# Autodesk Inventor assembly: Cabinet-LogicCircuit
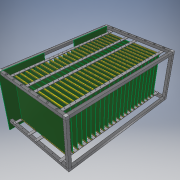
[picture p0: Inventor's stored thumbnail of the model, 180x180]
Saved by Autodesk Inventor 2018 (Build 220112000, 112)
## iProperties
Created: 2025-02-17
Part Number: Cabinet-LogicCircuit
Material: Všeobecné
Document SubType Name: Assembly
Designer: Jozko Mrkvicka
Author: Jozko Mrkvicka
## Documents named in this file (11)
- D:\05_Projekty\Projects_Inventor\Haluska9000\Cabinet-LogicCircuit.iam
- D:\05_Projekty\Projects_Inventor\Haluska9000\Profile-Connector.ipt
- D:\05_Projekty\Projects_Inventor\Haluska9000\Profile-Connector\Profile-Connector#15x15xCorner.ipt
- D:\05_Projekty\Projects_Inventor\Haluska9000\PCB.ipt
- D:\05_Projekty\Projects_Inventor\Haluska9000\CardGuideArray-4-Inch.iam
- D:\05_Projekty\Projects_Inventor\Haluska9000\CardGuideArray-6-Inch.iam
- D:\05_Projekty\Projects_Inventor\Haluska9000\Profile-Square-Gray\Profile-Square#Cabinet-LogicCircuit-Width.ipt
- D:\05_Projekty\Projects_Inventor\Haluska9000\Profile-Square-Gray\Profile-Square#Cabinet-LogicCircuit-Height.ipt
- D:\05_Projekty\Projects_Inventor\Haluska9000\Profile-Square-Gray\Profile-Square#Cabinet-LogicCircuit-Length.ipt
- D:\05_Projekty\Projects_Inventor\Haluska9000\Profile-Square-Gray.ipt
- D:\05_Projekty\Projects_Inventor\Haluska9000\PCB\PCB#LogicCircuit.ipt
## Components (49 placed, 8 different names)
1. Profile-Square#Cabinet-LogicCircuit-Width:15
2. Profile-Square#Cabinet-LogicCircuit-Width:18
3. Profile-Square#Cabinet-LogicCircuit-Width:21
4. Profile-Square#Cabinet-LogicCircuit-Width:24
5. Profile-Square#Cabinet-LogicCircuit-Height:14
6. Profile-Square#Cabinet-LogicCircuit-Height:17
7. Profile-Square#Cabinet-LogicCircuit-Height:20
8. Profile-Square#Cabinet-LogicCircuit-Height:23
9. Profile-Square#Cabinet-LogicCircuit-Length:13 — Stejný směr:152, Stejný směr:153, Proti sobě:353, Proti sobě:354, Proti sobě:356, Proti sobě:357
10. Profile-Square#Cabinet-LogicCircuit-Length:16 — Proti sobě:360, Proti sobě:361, Stejný směr:399, Stejný směr:400, Proti sobě:362, Proti sobě:363
11. Profile-Square#Cabinet-LogicCircuit-Length:19
12. Profile-Square#Cabinet-LogicCircuit-Length:22
13. Profile-Connector#15x15xCorner:17
14. Profile-Connector#15x15xCorner:18
15. Profile-Connector#15x15xCorner:19
16. Profile-Connector#15x15xCorner:20
17. Profile-Connector#15x15xCorner:21
18. Profile-Connector#15x15xCorner:22
19. Profile-Connector#15x15xCorner:23
20. Profile-Connector#15x15xCorner:24
21. PCB:19
22. PCB:20
23. CardGuideArray-4-Inch:1 [sub-assembly] — Stejný směr:152, Proti sobě:354, Proti sobě:357
24. CardGuideArray-6-Inch:1 [sub-assembly] — Stejný směr:153, Proti sobě:353, Proti sobě:356, Proti sobě:358, Proti sobě:359
25. PCB#LogicCircuit:1 — Stejný směr:154, Stejný směr:176, Stejný směr:360, Proti sobě:358, Proti sobě:359
26. PCB#LogicCircuit:2 — Stejný směr:154, Stejný směr:155, Stejný směr:176, Stejný směr:177, Stejný směr:360, Stejný směr:361
27. PCB#LogicCircuit:3 — Stejný směr:155, Stejný směr:156, Stejný směr:177, Stejný směr:178, Stejný směr:361, Stejný směr:362
28. PCB#LogicCircuit:4 — Stejný směr:156, Stejný směr:157, Stejný směr:178, Stejný směr:179, Stejný směr:362, Stejný směr:363
29. PCB#LogicCircuit:5 — Stejný směr:157, Stejný směr:158, Stejný směr:179, Stejný směr:359, Stejný směr:363, Stejný směr:364
30. PCB#LogicCircuit:6 — Stejný směr:158, Stejný směr:159, Stejný směr:359, Stejný směr:381, Stejný směr:364, Stejný směr:397
31. PCB#LogicCircuit:7 — Stejný směr:159, Stejný směr:160, Stejný směr:381, Stejný směr:365, Stejný směr:382, Stejný směr:397
32. PCB#LogicCircuit:8 — Stejný směr:160, Stejný směr:161, Stejný směr:365, Stejný směr:366, Stejný směr:382, Stejný směr:383
33. PCB#LogicCircuit:9 — Stejný směr:161, Stejný směr:162, Stejný směr:366, Stejný směr:367, Stejný směr:383, Stejný směr:384
34. PCB#LogicCircuit:10 — Stejný směr:162, Stejný směr:163, Stejný směr:367, Stejný směr:368, Stejný směr:384, Stejný směr:385
35. PCB#LogicCircuit:11 — Stejný směr:163, Stejný směr:164, Stejný směr:368, Stejný směr:369, Stejný směr:385, Stejný směr:386
36. PCB#LogicCircuit:12 — Stejný směr:164, Stejný směr:165, Stejný směr:369, Stejný směr:370, Stejný směr:386, Stejný směr:387
37. PCB#LogicCircuit:13 — Stejný směr:165, Stejný směr:166, Stejný směr:370, Stejný směr:371, Stejný směr:387, Stejný směr:388
38. PCB#LogicCircuit:14 — Stejný směr:166, Stejný směr:167, Stejný směr:371, Stejný směr:372, Stejný směr:388, Stejný směr:389
39. PCB#LogicCircuit:15 — Stejný směr:167, Stejný směr:168, Stejný směr:372, Stejný směr:373, Stejný směr:389, Stejný směr:390
40. PCB#LogicCircuit:16 — Stejný směr:168, Stejný směr:169, Stejný směr:373, Stejný směr:374, Stejný směr:390, Stejný směr:391
41. PCB#LogicCircuit:17 — Stejný směr:169, Stejný směr:170, Stejný směr:374, Stejný směr:375, Stejný směr:391, Stejný směr:392
42. PCB#LogicCircuit:18 — Stejný směr:170, Stejný směr:171, Stejný směr:375, Stejný směr:376, Stejný směr:392, Stejný směr:398
43. PCB#LogicCircuit:19 — Stejný směr:171, Stejný směr:172, Stejný směr:376, Stejný směr:377, Stejný směr:393, Stejný směr:398
44. PCB#LogicCircuit:20 — Stejný směr:172, Stejný směr:173, Stejný směr:377, Stejný směr:378, Stejný směr:393, Stejný směr:394
45. PCB#LogicCircuit:21 — Stejný směr:173, Stejný směr:174, Stejný směr:378, Stejný směr:379, Stejný směr:394, Stejný směr:395
46. PCB#LogicCircuit:22 — Stejný směr:174, Stejný směr:175, Stejný směr:379, Stejný směr:380, Stejný směr:395, Stejný směr:396
47. PCB#LogicCircuit:23 — Stejný směr:175, Stejný směr:380, Stejný směr:396
48. CardGuideArray-4-Inch:2 [sub-assembly] — Proti sobě:360, Stejný směr:399, Proti sobě:362
49. CardGuideArray-6-Inch:2 [sub-assembly] — Proti sobě:361, Stejný směr:400, Proti sobě:363
## Relationships (143: Flush 72, Mate 71)
- [Mate]: Profile-Square#Cabinet-LogicCircuit-Length:13 ↔ Profile-Connector#15x15xCorner:17
- [Mate]: Profile-Square#Cabinet-LogicCircuit-Length:13 ↔ Profile-Connector#15x15xCorner:17
- [Mate]: Profile-Square#Cabinet-LogicCircuit-Length:13 ↔ Profile-Connector#15x15xCorner:17
- [Mate]: Profile-Square#Cabinet-LogicCircuit-Height:14 ↔ Profile-Connector#15x15xCorner:17
- [Mate]: Profile-Square#Cabinet-LogicCircuit-Height:14 ↔ Profile-Connector#15x15xCorner:17
- [Mate]: Profile-Square#Cabinet-LogicCircuit-Height:14 ↔ Profile-Connector#15x15xCorner:17
- [Mate]: Profile-Square#Cabinet-LogicCircuit-Width:15 ↔ Profile-Connector#15x15xCorner:17
- [Mate]: Profile-Square#Cabinet-LogicCircuit-Width:15 ↔ Profile-Connector#15x15xCorner:17
- [Mate]: Profile-Square#Cabinet-LogicCircuit-Width:15 ↔ Profile-Connector#15x15xCorner:17
- [Mate]: Profile-Square#Cabinet-LogicCircuit-Length:13 ↔ Profile-Connector#15x15xCorner:18
- [Mate]: Profile-Square#Cabinet-LogicCircuit-Length:13 ↔ Profile-Connector#15x15xCorner:18
- [Mate]: Profile-Square#Cabinet-LogicCircuit-Length:13 ↔ Profile-Connector#15x15xCorner:18
- [Mate]: Profile-Square#Cabinet-LogicCircuit-Length:16 ↔ Profile-Connector#15x15xCorner:19
- [Mate]: Profile-Square#Cabinet-LogicCircuit-Length:16 ↔ Profile-Connector#15x15xCorner:19
- [Mate]: Profile-Square#Cabinet-LogicCircuit-Length:16 ↔ Profile-Connector#15x15xCorner:19
- [Mate]: Profile-Square#Cabinet-LogicCircuit-Height:17 ↔ Profile-Connector#15x15xCorner:19
- [Mate]: Profile-Square#Cabinet-LogicCircuit-Height:17 ↔ Profile-Connector#15x15xCorner:19
- [Mate]: Profile-Square#Cabinet-LogicCircuit-Height:17 ↔ Profile-Connector#15x15xCorner:19
- [Mate]: Profile-Square#Cabinet-LogicCircuit-Width:18 ↔ Profile-Connector#15x15xCorner:19
- [Mate]: Profile-Square#Cabinet-LogicCircuit-Width:18 ↔ Profile-Connector#15x15xCorner:19
- [Mate]: Profile-Square#Cabinet-LogicCircuit-Width:18 ↔ Profile-Connector#15x15xCorner:19
- [Mate]: Profile-Square#Cabinet-LogicCircuit-Length:16 ↔ Profile-Connector#15x15xCorner:20
- [Mate]: Profile-Square#Cabinet-LogicCircuit-Length:16 ↔ Profile-Connector#15x15xCorner:20
- [Mate]: Profile-Square#Cabinet-LogicCircuit-Length:16 ↔ Profile-Connector#15x15xCorner:20
- [Mate]: Profile-Square#Cabinet-LogicCircuit-Height:17 ↔ Profile-Connector#15x15xCorner:18
- [Mate]: Profile-Square#Cabinet-LogicCircuit-Height:17 ↔ Profile-Connector#15x15xCorner:18
- [Mate]: Profile-Square#Cabinet-LogicCircuit-Height:17 ↔ Profile-Connector#15x15xCorner:18
- [Mate]: Profile-Square#Cabinet-LogicCircuit-Length:19 ↔ Profile-Connector#15x15xCorner:21
- [Mate]: Profile-Square#Cabinet-LogicCircuit-Length:19 ↔ Profile-Connector#15x15xCorner:21
- [Mate]: Profile-Square#Cabinet-LogicCircuit-Length:19 ↔ Profile-Connector#15x15xCorner:21
- [Mate]: Profile-Square#Cabinet-LogicCircuit-Height:20 ↔ Profile-Connector#15x15xCorner:21
- [Mate]: Profile-Square#Cabinet-LogicCircuit-Height:20 ↔ Profile-Connector#15x15xCorner:21
- [Mate]: Profile-Square#Cabinet-LogicCircuit-Height:20 ↔ Profile-Connector#15x15xCorner:21
- [Mate]: Profile-Square#Cabinet-LogicCircuit-Width:21 ↔ Profile-Connector#15x15xCorner:21
- [Mate]: Profile-Square#Cabinet-LogicCircuit-Width:21 ↔ Profile-Connector#15x15xCorner:21
- [Mate]: Profile-Square#Cabinet-LogicCircuit-Width:21 ↔ Profile-Connector#15x15xCorner:21
- [Mate]: Profile-Square#Cabinet-LogicCircuit-Length:19 ↔ Profile-Connector#15x15xCorner:22
- [Mate]: Profile-Square#Cabinet-LogicCircuit-Length:19 ↔ Profile-Connector#15x15xCorner:22
- [Mate]: Profile-Square#Cabinet-LogicCircuit-Length:19 ↔ Profile-Connector#15x15xCorner:22
- [Mate]: Profile-Square#Cabinet-LogicCircuit-Length:22 ↔ Profile-Connector#15x15xCorner:23
- [Mate]: Profile-Square#Cabinet-LogicCircuit-Length:22 ↔ Profile-Connector#15x15xCorner:23
- [Mate]: Profile-Square#Cabinet-LogicCircuit-Length:22 ↔ Profile-Connector#15x15xCorner:23
- [Mate]: Profile-Square#Cabinet-LogicCircuit-Height:23 ↔ Profile-Connector#15x15xCorner:23
- [Mate]: Profile-Square#Cabinet-LogicCircuit-Height:23 ↔ Profile-Connector#15x15xCorner:23
- [Mate]: Profile-Square#Cabinet-LogicCircuit-Height:23 ↔ Profile-Connector#15x15xCorner:23
- [Mate]: Profile-Square#Cabinet-LogicCircuit-Width:24 ↔ Profile-Connector#15x15xCorner:23
- [Mate]: Profile-Square#Cabinet-LogicCircuit-Width:24 ↔ Profile-Connector#15x15xCorner:23
- [Mate]: Profile-Square#Cabinet-LogicCircuit-Width:24 ↔ Profile-Connector#15x15xCorner:23
- [Mate]: Profile-Square#Cabinet-LogicCircuit-Length:22 ↔ Profile-Connector#15x15xCorner:24
- [Mate]: Profile-Square#Cabinet-LogicCircuit-Length:22 ↔ Profile-Connector#15x15xCorner:24
- [Mate]: Profile-Square#Cabinet-LogicCircuit-Length:22 ↔ Profile-Connector#15x15xCorner:24
- [Mate]: Profile-Square#Cabinet-LogicCircuit-Height:23 ↔ Profile-Connector#15x15xCorner:22
- [Mate]: Profile-Square#Cabinet-LogicCircuit-Height:23 ↔ Profile-Connector#15x15xCorner:22
- [Mate]: Profile-Square#Cabinet-LogicCircuit-Height:23 ↔ Profile-Connector#15x15xCorner:22
- [Mate]: Profile-Square#Cabinet-LogicCircuit-Width:21 ↔ Profile-Connector#15x15xCorner:18
- [Mate]: Profile-Square#Cabinet-LogicCircuit-Width:21 ↔ Profile-Connector#15x15xCorner:18
- [Mate]: Profile-Square#Cabinet-LogicCircuit-Width:21 ↔ Profile-Connector#15x15xCorner:18
- [Flush]: Profile-Square#Cabinet-LogicCircuit-Width:18 ↔ PCB:19
- [Mate]: Profile-Square#Cabinet-LogicCircuit-Width:18 ↔ PCB:19
- [Mate]: Profile-Square#Cabinet-LogicCircuit-Length:16 ↔ PCB:19
- [Mate]: Profile-Square#Cabinet-LogicCircuit-Width:18 ↔ PCB:20
- [Flush]: Profile-Square#Cabinet-LogicCircuit-Width:18 ↔ PCB:20
- [Mate]: Profile-Square#Cabinet-LogicCircuit-Length:22 ↔ PCB:20
- Stejný směr:152 [Flush]: Profile-Square#Cabinet-LogicCircuit-Length:13 ↔ CardGuideArray-4-Inch:1
- Stejný směr:153 [Flush]: Profile-Square#Cabinet-LogicCircuit-Length:13 ↔ CardGuideArray-6-Inch:1
- Proti sobě:353 [Mate]: Profile-Square#Cabinet-LogicCircuit-Length:13 ↔ CardGuideArray-6-Inch:1
- Proti sobě:354 [Mate]: Profile-Square#Cabinet-LogicCircuit-Length:13 ↔ CardGuideArray-4-Inch:1
- Proti sobě:356 [Mate]: Profile-Square#Cabinet-LogicCircuit-Length:13 ↔ CardGuideArray-6-Inch:1
- Proti sobě:357 [Mate]: Profile-Square#Cabinet-LogicCircuit-Length:13 ↔ CardGuideArray-4-Inch:1
- Stejný směr:154 [Flush] (25.4 mm): PCB#LogicCircuit:1 ↔ PCB#LogicCircuit:2
- Stejný směr:155 [Flush] (25.4 mm): PCB#LogicCircuit:2 ↔ PCB#LogicCircuit:3
- Stejný směr:156 [Flush] (25.4 mm): PCB#LogicCircuit:3 ↔ PCB#LogicCircuit:4
- Stejný směr:157 [Flush] (25.4 mm): PCB#LogicCircuit:4 ↔ PCB#LogicCircuit:5
- Stejný směr:158 [Flush] (25.4 mm): PCB#LogicCircuit:5 ↔ PCB#LogicCircuit:6
- Stejný směr:159 [Flush] (25.4 mm): PCB#LogicCircuit:6 ↔ PCB#LogicCircuit:7
- Stejný směr:160 [Flush] (25.4 mm): PCB#LogicCircuit:7 ↔ PCB#LogicCircuit:8
- Stejný směr:161 [Flush] (25.4 mm): PCB#LogicCircuit:8 ↔ PCB#LogicCircuit:9
- Stejný směr:162 [Flush] (25.4 mm): PCB#LogicCircuit:9 ↔ PCB#LogicCircuit:10
- Stejný směr:163 [Flush] (25.4 mm): PCB#LogicCircuit:10 ↔ PCB#LogicCircuit:11
- Stejný směr:164 [Flush] (25.4 mm): PCB#LogicCircuit:11 ↔ PCB#LogicCircuit:12
- Stejný směr:165 [Flush] (25.4 mm): PCB#LogicCircuit:12 ↔ PCB#LogicCircuit:13
- Stejný směr:166 [Flush] (25.4 mm): PCB#LogicCircuit:13 ↔ PCB#LogicCircuit:14
- Stejný směr:167 [Flush] (25.4 mm): PCB#LogicCircuit:14 ↔ PCB#LogicCircuit:15
- Stejný směr:168 [Flush] (25.4 mm): PCB#LogicCircuit:15 ↔ PCB#LogicCircuit:16
- Stejný směr:169 [Flush] (25.4 mm): PCB#LogicCircuit:16 ↔ PCB#LogicCircuit:17
- Stejný směr:170 [Flush] (25.4 mm): PCB#LogicCircuit:17 ↔ PCB#LogicCircuit:18
- Stejný směr:171 [Flush] (25.4 mm): PCB#LogicCircuit:18 ↔ PCB#LogicCircuit:19
- Stejný směr:172 [Flush] (25.4 mm): PCB#LogicCircuit:19 ↔ PCB#LogicCircuit:20
- Stejný směr:173 [Flush] (25.4 mm): PCB#LogicCircuit:20 ↔ PCB#LogicCircuit:21
- Stejný směr:174 [Flush] (25.4 mm): PCB#LogicCircuit:21 ↔ PCB#LogicCircuit:22
- Stejný směr:175 [Flush] (25.4 mm): PCB#LogicCircuit:22 ↔ PCB#LogicCircuit:23
- Stejný směr:176 [Flush]: PCB#LogicCircuit:1 ↔ PCB#LogicCircuit:2
- Stejný směr:177 [Flush]: PCB#LogicCircuit:2 ↔ PCB#LogicCircuit:3
- Stejný směr:178 [Flush]: PCB#LogicCircuit:3 ↔ PCB#LogicCircuit:4
- Stejný směr:179 [Flush]: PCB#LogicCircuit:4 ↔ PCB#LogicCircuit:5
- Stejný směr:359 [Flush]: PCB#LogicCircuit:5 ↔ PCB#LogicCircuit:6
- Stejný směr:381 [Flush]: PCB#LogicCircuit:6 ↔ PCB#LogicCircuit:7
- Stejný směr:360 [Flush]: PCB#LogicCircuit:1 ↔ PCB#LogicCircuit:2
- Stejný směr:361 [Flush]: PCB#LogicCircuit:2 ↔ PCB#LogicCircuit:3
- Stejný směr:362 [Flush]: PCB#LogicCircuit:3 ↔ PCB#LogicCircuit:4
- Stejný směr:363 [Flush]: PCB#LogicCircuit:4 ↔ PCB#LogicCircuit:5
- Stejný směr:364 [Flush]: PCB#LogicCircuit:5 ↔ PCB#LogicCircuit:6
- Stejný směr:365 [Flush]: PCB#LogicCircuit:7 ↔ PCB#LogicCircuit:8
- Stejný směr:366 [Flush]: PCB#LogicCircuit:8 ↔ PCB#LogicCircuit:9
- Stejný směr:367 [Flush]: PCB#LogicCircuit:9 ↔ PCB#LogicCircuit:10
- Stejný směr:368 [Flush]: PCB#LogicCircuit:10 ↔ PCB#LogicCircuit:11
- Stejný směr:369 [Flush]: PCB#LogicCircuit:11 ↔ PCB#LogicCircuit:12
- Stejný směr:370 [Flush]: PCB#LogicCircuit:12 ↔ PCB#LogicCircuit:13
- Stejný směr:371 [Flush]: PCB#LogicCircuit:13 ↔ PCB#LogicCircuit:14
- Stejný směr:372 [Flush]: PCB#LogicCircuit:14 ↔ PCB#LogicCircuit:15
- Stejný směr:373 [Flush]: PCB#LogicCircuit:15 ↔ PCB#LogicCircuit:16
- Stejný směr:374 [Flush]: PCB#LogicCircuit:16 ↔ PCB#LogicCircuit:17
- Stejný směr:375 [Flush]: PCB#LogicCircuit:17 ↔ PCB#LogicCircuit:18
- Stejný směr:376 [Flush]: PCB#LogicCircuit:18 ↔ PCB#LogicCircuit:19
- Stejný směr:377 [Flush]: PCB#LogicCircuit:19 ↔ PCB#LogicCircuit:20
- Stejný směr:378 [Flush]: PCB#LogicCircuit:20 ↔ PCB#LogicCircuit:21
- Stejný směr:379 [Flush]: PCB#LogicCircuit:21 ↔ PCB#LogicCircuit:22
- Stejný směr:380 [Flush]: PCB#LogicCircuit:22 ↔ PCB#LogicCircuit:23
- Stejný směr:382 [Flush]: PCB#LogicCircuit:7 ↔ PCB#LogicCircuit:8
- Stejný směr:383 [Flush]: PCB#LogicCircuit:8 ↔ PCB#LogicCircuit:9
- Stejný směr:384 [Flush]: PCB#LogicCircuit:9 ↔ PCB#LogicCircuit:10
- Stejný směr:385 [Flush]: PCB#LogicCircuit:10 ↔ PCB#LogicCircuit:11
- Stejný směr:386 [Flush]: PCB#LogicCircuit:11 ↔ PCB#LogicCircuit:12
- Stejný směr:387 [Flush]: PCB#LogicCircuit:12 ↔ PCB#LogicCircuit:13
- Stejný směr:388 [Flush]: PCB#LogicCircuit:13 ↔ PCB#LogicCircuit:14
- Stejný směr:389 [Flush]: PCB#LogicCircuit:14 ↔ PCB#LogicCircuit:15
- Stejný směr:390 [Flush]: PCB#LogicCircuit:15 ↔ PCB#LogicCircuit:16
- Stejný směr:391 [Flush]: PCB#LogicCircuit:16 ↔ PCB#LogicCircuit:17
- Stejný směr:392 [Flush]: PCB#LogicCircuit:17 ↔ PCB#LogicCircuit:18
- Stejný směr:393 [Flush]: PCB#LogicCircuit:19 ↔ PCB#LogicCircuit:20
- Stejný směr:394 [Flush]: PCB#LogicCircuit:20 ↔ PCB#LogicCircuit:21
- Stejný směr:395 [Flush]: PCB#LogicCircuit:21 ↔ PCB#LogicCircuit:22
- Stejný směr:396 [Flush]: PCB#LogicCircuit:22 ↔ PCB#LogicCircuit:23
- Stejný směr:397 [Flush]: PCB#LogicCircuit:6 ↔ PCB#LogicCircuit:7
- Stejný směr:398 [Flush]: PCB#LogicCircuit:18 ↔ PCB#LogicCircuit:19
- Proti sobě:358 [Mate]: CardGuideArray-6-Inch:1 ↔ PCB#LogicCircuit:1
- Proti sobě:359 [Mate]: CardGuideArray-6-Inch:1 ↔ PCB#LogicCircuit:1
- Proti sobě:360 [Mate]: Profile-Square#Cabinet-LogicCircuit-Length:16 ↔ CardGuideArray-4-Inch:2
- Proti sobě:361 [Mate]: Profile-Square#Cabinet-LogicCircuit-Length:16 ↔ CardGuideArray-6-Inch:2
- Stejný směr:399 [Flush]: Profile-Square#Cabinet-LogicCircuit-Length:16 ↔ CardGuideArray-4-Inch:2
- Stejný směr:400 [Flush]: Profile-Square#Cabinet-LogicCircuit-Length:16 ↔ CardGuideArray-6-Inch:2
- Proti sobě:362 [Mate]: Profile-Square#Cabinet-LogicCircuit-Length:16 ↔ CardGuideArray-4-Inch:2
- Proti sobě:363 [Mate]: Profile-Square#Cabinet-LogicCircuit-Length:16 ↔ CardGuideArray-6-Inch:2
## Named parameters: d418_d182 = 0 mm, d419_d183 = 0 mm, d420_d184 = 0 mm, d445_d179 = 0 mm, d446_d180 = 0 mm, d447_d181 = 0 mm, d485_d297 = 0 mm, d486_d298 = 0 mm, d487_d299 = 0 mm, d490_d245 = 0 mm, d491_d246 = 0 mm, d492_d247 = 0 mm, d493_d248 = 0 mm, d494_d249 = 0 mm, d495_d250 = 0 mm, d496_d251 = 0 mm, d497_d252 = 0 mm, d498_d253 = 0 mm, d499_d254 = 0 mm, d500_d255_d243 = 0 mm, d501_d256_d244 = 0 mm, d502_d257_d245 = 0 mm, d503_d258_d246 = 0 mm, d504_d259_d247 = 0 mm, d505_d260_d248 = 0 mm, d506_d261_d249 = 0 mm, d507_d262_d250 = 0 mm, d508_d263_d251 = 0 mm, d509_d264_d252 = 0 mm, d510_d265_d253 = 0 mm, d511_d266_d254 = 0 mm, d512_d267 = 0 mm, d513_d268 = 0 mm, d514_d269 = 0 mm, d515_d270_d260_d248 = 0 mm, d516_d271_d261_d249 = 0 mm, d517_d272_d262_d250 = 0 mm, d518_d273_d263_d251 = 0 mm, d519_d274_d264_d252 = 0 mm, d520_d275_d265_d253 = 0 mm, d521_d276_d266_d254 = 0 mm, d522_d277_d267 = 0 mm, d523_d278_d268 = 0 mm, d524_d279_d269 = 0 mm, d525_d280_d243 = 0 mm, d526_d281_d244 = 0 mm, d527_d282_d245 = 0 mm, d528_d283_d246 = 0 mm, d529_d284_d247 = 0 mm, d530_d285_d248 = 0 mm, d531_d286_d249 = 0 mm, d532_d287_d250 = 0 mm, d533_d288_d251 = 0 mm, d534_d289_d252 = 0 mm, d535_d290_d253 = 0 mm, d536_d291_d254 = 0 mm, d537_d292_d255_d243 = 0 mm, d538_d293_d256_d244 = 0 mm, d539_d294_d257_d245 = 0 mm, d540_d295_d258_d246 = 0 mm, d541_d296_d259_d247 = 0 mm, d542_d243 = 0 mm, d543_d244 = 0 mm
